# Autodesk Inventor assembly: 5
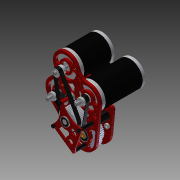
[picture p0: Inventor's stored thumbnail of the model, 180x180]
Saved by Autodesk Inventor 2013 (Build 170138000, 138)
## iProperties
Created: 2013-07-09
Part Number: 5
Document SubType Name: Assembly
Designer: mvarma
Author: mvarma
## Documents named in this file (40)
- C:\Users\mvarma\Desktop\GRT 2013-2014 Gearbox\Mark 5\Mark 5 Rendering Copy.iam
- C:\Users\mvarma\Desktop\GRT 2013-2014 Gearbox\Mark 5\Plates\Mounting Plate\Mounting Plate.ipt
- C:\Users\mvarma\Desktop\GRT 2013-2014 Gearbox\Mark 5\Plates\Cim Plate\Cim Plate.ipt
- C:\Users\mvarma\Desktop\GRT 2013-2014 Gearbox\Mark 5\Plates\Main Connecting Standoff Thick.ipt
- C:\Users\mvarma\Desktop\GRT 2013-2014 Gearbox\Mark 5\Plates\Main Connecting Standoff Thin.ipt
- C:\Users\mvarma\Desktop\GRT 2013-2014 Gearbox\Mark 5\Bearings\FR8-2RS.ipt
- C:\Users\mvarma\Desktop\GRT 2013-2014 Gearbox\Mark 5\Bearings\FR6-2RS.ipt
- C:\Users\mvarma\Desktop\GRT 2013-2014 Gearbox\Mark 5\Shafts\Cluster Shaft\15T 20DP - .375 Hex Bore.ipt
- C:\Users\mvarma\Desktop\GRT 2013-2014 Gearbox\Mark 5\Shafts\Cluster Shaft\28T 20DP - .375 Hex Bore.ipt
- C:\Users\mvarma\Desktop\GRT 2013-2014 Gearbox\Mark 5\Shafts\Cluster Shaft\Cluster Shaft Spacer.ipt
- C:\Users\mvarma\Desktop\GRT 2013-2014 Gearbox\Mark 5\Shafts\Cluster Shaft\Cluster Shaft.ipt
- C:\Users\mvarma\Desktop\GRT 2013-2014 Gearbox\Mark 5\Shafts\Cluster Shaft\48T 3mm GT2 - .375 Hex Broach - Hubless.ipt
- C:\Users\mvarma\Desktop\GRT 2013-2014 Gearbox\Mark 5\Shafts\Cluster Shaft\Flexible Shaft Coupler 6208K411.ipt
- C:\Users\mvarma\Desktop\GRT 2013-2014 Gearbox\Mark 5\Encoder\Encoder Mount.ipt
- C:\Users\mvarma\Desktop\GRT 2013-2014 Gearbox\Mark 5\Encoder\S4-120-250-N-S-B.ipt
- C:\Users\mvarma\Desktop\GRT 2013-2014 Gearbox\Mark 5\Shafts\Output Shaft\Output Shaft Hex Sleave.ipt
- C:\Users\mvarma\Desktop\GRT 2013-2014 Gearbox\Mark 5\Shafts\Output Shaft\Output Shaft Insert.ipt
- C:\Users\mvarma\Desktop\GRT 2013-2014 Gearbox\Mark 5\Shafts\Output Shaft\Output Shaft.ipt
- C:\Users\mvarma\Desktop\GRT 2013-2014 Gearbox\Mark 5\Shafts\Output Shaft\35T 20DP - .188 Ball Shifting Bore.ipt
- C:\Users\mvarma\Desktop\GRT 2013-2014 Gearbox\Mark 5\Shafts\Output Shaft\48T 20DP - .188 Ball Shifting Bore.ipt
- C:\Users\mvarma\Desktop\GRT 2013-2014 Gearbox\Mark 5\Bearings\Thrust Bearing Washer - .6250 Bore.ipt
- C:\Users\mvarma\Desktop\GRT 2013-2014 Gearbox\Mark 5\Bearings\R10-Open.ipt
- C:\Users\mvarma\Desktop\GRT 2013-2014 Gearbox\Mark 5\Shafts\Output Shaft\Shim 10 thou .500 Bore.ipt
- C:\Users\mvarma\Desktop\GRT 2013-2014 Gearbox\Mark 5\Shafts\Output Shaft\Shim 10 thou .625 Bore.ipt
- C:\Users\mvarma\Desktop\GRT 2013-2014 Gearbox\Mark 5\Plates\Mounting Plate\10-32 Clinch Style Pem Nut .091 Minimum Panel Thickness.ipt
- C:\Users\mvarma\Desktop\GRT 2013-2014 Gearbox\Mark 5\Plates\Mounting Plate\.25-20 Clinch Style Pem Nut .125 Minimum Panel Thickness.ipt
- C:\Users\mvarma\Desktop\GRT 2013-2014 Gearbox\Mark 5\Motors\CIM Can.ipt
- C:\Users\mvarma\Desktop\GRT 2013-2014 Gearbox\Mark 5\Motors\Rotor.ipt
- C:\Users\mvarma\Desktop\GRT 2013-2014 Gearbox\Mark 5\Motors\Mini CIM Can.ipt
- C:\Users\mvarma\Desktop\GRT 2013-2014 Gearbox\Mark 5\Pulleys\16T 3mm GT2 - 8mm Key Broach.ipt
- C:\Users\mvarma\Desktop\GRT 2013-2014 Gearbox\Mark 5\Belts\267 mm Belt.ipt
- C:\Users\mvarma\Desktop\GRT 2013-2014 Gearbox\Mark 5\Belts\285 mm Belt.ipt
- C:\Users\mvarma\Desktop\GRT 2013-2014 Gearbox\Mark 5\Plates\Tensioning Shaft.ipt
- C:\Users\mvarma\Desktop\GRT 2013-2014 Gearbox\Mark 5\Plates\Belt Shaft Spacer 2.ipt
- C:\Users\mvarma\Desktop\GRT 2013-2014 Gearbox\Mark 5\Bearings\R4-2RS.ipt
- C:\Users\mvarma\Desktop\GRT 2013-2014 Gearbox\Mark 5\Shafts\Cluster Shaft\Shim 10 thou .375 Bore.ipt
- C:\Users\mvarma\Desktop\GRT 2013-2014 Gearbox\Mark 5\Plates\Pnuematic Plate.ipt
- C:\Users\mvarma\Desktop\GRT 2013-2014 Gearbox\Mark 5\Plates\Supporting Plate Standoff Long.ipt
- C:\Users\mvarma\Desktop\GRT 2013-2014 Gearbox\Mark 5\Plates\Supporting Plate Standoff Short.ipt
- C:\Users\mvarma\Desktop\GRT 2013-2014 Gearbox\Mark 5\Bolts\Socket Head Cap Screw 10-32 Thread 3.000 Length.ipt
## Components (57 placed, 39 different names)
1. Mounting Plate:1 — Mate:1, Mate:2, Mate:3, Mate:5, Mate:11, Mate:13, Mate:15, Mate:16, Mate:17, Mate:18, Mate:52, Mate:53, Mate:54, Mate:76, Mate:77, Mate:78, Mate:79, Mate:80, Mate:81, Mate:82, Mate:83, Mate:101, Mate:102
2. Cim Plate:1 — Mate:7, Mate:8, Mate:9, Mate:12, Mate:14, Mate:19, Mate:86, Mate:87, Mate:88, Mate:89, Mate:90, Mate:91, Mate:96, Mate:97, Mate:98, Mate:115, Mate:116, Mate:124, Mate:125, Mate:126, Mate:130, Mate:131, Mate:132, Mate:133, Mate:134, Mate:135
3. Main Connecting Standoff Thick:1 — Mate:5, Mate:8, Mate:18
4. Main Connecting Standoff Thick:2 — Mate:3, Mate:7, Mate:17, Mate:19
5. Main Connecting Standoff Thin:1 — Mate:1, Mate:2, Mate:9
6. FR8-2RS:1 — Mate:12, Mate:14, Mate:55, Mate:75
7. FR8-2RS:2 — Mate:11, Mate:13
8. FR6-2RS:1 — Mate:15, Mate:16, Mate:33
9. 15T 20DP - .375 Hex Bore:1 — Mate:34, Mate:36, Mate:45, Mate:144
10. 28T 20DP - .375 Hex Bore:1 — Mate:34, Mate:37, Mate:38, Mate:45
11. Cluster Shaft Spacer:1 — Mate:30, Mate:31, Mate:33, Mate:38
12. Cluster Shaft:1 — Mate:30, Mate:31, Mate:36, Mate:37, Mate:39, Mate:40, Mate:41, Mate:42, Mate:44, Mate:48, Mate:49, Mate:121, Mate:123
13. 48T 3mm GT2 - .375 Hex Broach - Hubless:1 — Mate:39, Mate:41, Mate:43, Mate:44, Mate:104, Mate:106
14. 48T 3mm GT2 - .375 Hex Broach - Hubless:2 — Mate:40, Mate:42, Mate:43, Mate:108, Mate:122
15. Flexible Shaft Coupler 6208K411:1 — Mate:48, Mate:49
16. Encoder Mount:1 — Mate:50, Mate:51, Mate:52, Mate:53, Mate:54
17. S4-120-250-N-S-B:1 — Mate:50, Mate:51
18. Output Shaft Hex Sleave:1 — Mate:58, Mate:59, Flush:1
19. Output Shaft Insert:1 — Mate:56, Mate:57
20. Output Shaft:1 — Mate:55, Mate:56, Mate:57, Mate:58, Mate:59, Flush:1, Mate:61, Mate:66, Mate:67, Mate:70, Flush:2, Mate:72, Mate:73, Mate:75
21. 35T 20DP - .188 Ball Shifting Bore:1 — Mate:60, Mate:61, Mate:64, Mate:65, Mate:68
22. 48T 20DP - .188 Ball Shifting Bore:1 — Mate:60, Mate:62, Mate:63, Mate:69
23. Thrust Bearing Washer - .6250 Bore:1 — Mate:67, Mate:69, Mate:71
24. Thrust Bearing Washer - .6250 Bore:2 — Mate:66, Mate:68, Mate:74
25. R10-Open:1 — Mate:62, Mate:63, Mate:74
26. R10-Open:2 — Mate:64, Mate:65
27. Shim 10 thou .500 Bore:1 — Mate:72, Mate:73
28. Shim 10 thou .625 Bore:1 — Mate:70, Mate:71, Flush:2
29. 10-32 Clinch Style Pem Nut .091 Minimum Panel Thickness:1 — Mate:77, Mate:80
30. 10-32 Clinch Style Pem Nut .091 Minimum Panel Thickness:2 — Mate:78, Mate:81
31. 10-32 Clinch Style Pem Nut .091 Minimum Panel Thickness:3 — Mate:76, Mate:79
32. .25-20 Clinch Style Pem Nut .125 Minimum Panel Thickness:1 — Mate:82, Mate:101
33. .25-20 Clinch Style Pem Nut .125 Minimum Panel Thickness:2 — Mate:83, Mate:102
34. CIM Can:1 — Mate:88, Mate:89, Mate:90, Mate:94, Mate:95
35. CIM Can:2 — Mate:86, Mate:87, Mate:91, Mate:92, Mate:93
36. Rotor:1 — Mate:94, Mate:95, Mate:105, Mate:109
37. Rotor:2 — Mate:92, Mate:93, Mate:103
38. Rotor:3 — Mate:99, Mate:100, Mate:107, Mate:112
39. Mini CIM Can:1 — Mate:96, Mate:97, Mate:98, Mate:99, Mate:100
40. 16T 3mm GT2 - 8mm Key Broach:1 — Mate:105, Mate:106, Flush:3
41. 16T 3mm GT2 - 8mm Key Broach:2 — Mate:107, Mate:108, Mate:113
42. 16T 3mm GT2 - 8mm Key Broach:3 — Mate:103, Mate:104
43. 267 mm Belt:1 — Mate:109, Flush:3, Mate:143
44. 285 mm Belt:1 — Mate:112, Mate:113, Mate:142
45. Tensioning Shaft:1 — Mate:114, Flush:4, Mate:115, Mate:116, Mate:119, Mate:120
46. Belt Shaft Spacer 2:1 — Mate:114, Flush:4
47. R4-2RS:1 — Mate:117, Mate:118, Mate:119
48. R4-2RS:2 — Mate:117, Mate:118, Mate:120
49. Shim 10 thou .375 Bore:1 — Mate:121, Mate:122, Mate:129
50. Pnuematic Plate:1 — Mate:123, Mate:124, Mate:125, Mate:126, Mate:127, Mate:128, Mate:136, Mate:137, Mate:138, Mate:139, Mate:140, Mate:141, Mate:142, Mate:143, Mate:144
51. FR6-2RS:2 — Mate:127, Mate:128, Mate:129
52. Supporting Plate Standoff Long:1 — Mate:131, Mate:132
53. Supporting Plate Standoff Long:2 — Mate:130, Mate:133
54. Supporting Plate Standoff Short:1 — Mate:134, Mate:135
55. Socket Head Cap Screw 10-32 Thread 3.000 Length:1 — Mate:138, Mate:141
56. Socket Head Cap Screw 10-32 Thread 3.000 Length:2 — Mate:137, Mate:140
57. Socket Head Cap Screw 10-32 Thread 3.000 Length:3 — Mate:136, Mate:139
## Relationships (127: Mate 123, Flush 4)
- Mate:1: Mounting Plate:1 ↔ Main Connecting Standoff Thin:1
- Mate:2: Mounting Plate:1 ↔ Main Connecting Standoff Thin:1
- Mate:3: Mounting Plate:1 ↔ Main Connecting Standoff Thick:2
- Mate:5: Mounting Plate:1 ↔ Main Connecting Standoff Thick:1
- Mate:7: Cim Plate:1 ↔ Main Connecting Standoff Thick:2
- Mate:8: Cim Plate:1 ↔ Main Connecting Standoff Thick:1
- Mate:9: Cim Plate:1 ↔ Main Connecting Standoff Thin:1
- Mate:11: Mounting Plate:1 ↔ FR8-2RS:2
- Mate:12: Cim Plate:1 ↔ FR8-2RS:1
- Mate:13: Mounting Plate:1 ↔ FR8-2RS:2
- Mate:14: Cim Plate:1 ↔ FR8-2RS:1
- Mate:15: Mounting Plate:1 ↔ FR6-2RS:1
- Mate:16: Mounting Plate:1 ↔ FR6-2RS:1
- Mate:17: Mounting Plate:1 ↔ Main Connecting Standoff Thick:2
- Mate:18: Mounting Plate:1 ↔ Main Connecting Standoff Thick:1
- Mate:19: Cim Plate:1 ↔ Main Connecting Standoff Thick:2
- Mate:30: Cluster Shaft Spacer:1 ↔ Cluster Shaft:1
- Mate:31: Cluster Shaft Spacer:1 ↔ Cluster Shaft:1
- Mate:33: FR6-2RS:1 ↔ Cluster Shaft Spacer:1
- Mate:34: 15T 20DP - .375 Hex Bore:1 ↔ 28T 20DP - .375 Hex Bore:1
- Mate:36: 15T 20DP - .375 Hex Bore:1 ↔ Cluster Shaft:1
- Mate:37: 28T 20DP - .375 Hex Bore:1 ↔ Cluster Shaft:1
- Mate:38: 28T 20DP - .375 Hex Bore:1 ↔ Cluster Shaft Spacer:1
- Mate:39: Cluster Shaft:1 ↔ 48T 3mm GT2 - .375 Hex Broach - Hubless:1
- Mate:40: Cluster Shaft:1 ↔ 48T 3mm GT2 - .375 Hex Broach - Hubless:2
- Mate:41: Cluster Shaft:1 ↔ 48T 3mm GT2 - .375 Hex Broach - Hubless:1
- Mate:42: Cluster Shaft:1 ↔ 48T 3mm GT2 - .375 Hex Broach - Hubless:2
- Mate:43: 48T 3mm GT2 - .375 Hex Broach - Hubless:1 ↔ 48T 3mm GT2 - .375 Hex Broach - Hubless:2
- Mate:44: Cluster Shaft:1 ↔ 48T 3mm GT2 - .375 Hex Broach - Hubless:1
- Mate:45: 15T 20DP - .375 Hex Bore:1 ↔ 28T 20DP - .375 Hex Bore:1
- Mate:48: Cluster Shaft:1 ↔ Flexible Shaft Coupler 6208K411:1
- Mate:49: Cluster Shaft:1 ↔ Flexible Shaft Coupler 6208K411:1
- Mate:50: Encoder Mount:1 ↔ S4-120-250-N-S-B:1
- Mate:51: Encoder Mount:1 ↔ S4-120-250-N-S-B:1
- Mate:52: Mounting Plate:1 ↔ Encoder Mount:1
- Mate:53: Mounting Plate:1 ↔ Encoder Mount:1
- Mate:54: Mounting Plate:1 ↔ Encoder Mount:1
- Mate:55: FR8-2RS:1 ↔ Output Shaft:1
- Mate:56: Output Shaft Insert:1 ↔ Output Shaft:1
- Mate:57: Output Shaft Insert:1 ↔ Output Shaft:1
- Mate:58: Output Shaft Hex Sleave:1 ↔ Output Shaft:1
- Mate:59: Output Shaft Hex Sleave:1 ↔ Output Shaft:1
- Flush:1: Output Shaft Hex Sleave:1 ↔ Output Shaft:1
- Mate:60: 35T 20DP - .188 Ball Shifting Bore:1 ↔ 48T 20DP - .188 Ball Shifting Bore:1
- Mate:61: Output Shaft:1 ↔ 35T 20DP - .188 Ball Shifting Bore:1
- Mate:62: 48T 20DP - .188 Ball Shifting Bore:1 ↔ R10-Open:1
- Mate:63: 48T 20DP - .188 Ball Shifting Bore:1 ↔ R10-Open:1
- Mate:64: 35T 20DP - .188 Ball Shifting Bore:1 ↔ R10-Open:2
- Mate:65: 35T 20DP - .188 Ball Shifting Bore:1 ↔ R10-Open:2
- Mate:66: Output Shaft:1 ↔ Thrust Bearing Washer - .6250 Bore:2
- Mate:67: Output Shaft:1 ↔ Thrust Bearing Washer - .6250 Bore:1
- Mate:68: 35T 20DP - .188 Ball Shifting Bore:1 ↔ Thrust Bearing Washer - .6250 Bore:2
- Mate:69: 48T 20DP - .188 Ball Shifting Bore:1 ↔ Thrust Bearing Washer - .6250 Bore:1
- Mate:70: Output Shaft:1 ↔ Shim 10 thou .625 Bore:1
- Mate:71: Thrust Bearing Washer - .6250 Bore:1 ↔ Shim 10 thou .625 Bore:1
- Flush:2: Output Shaft:1 ↔ Shim 10 thou .625 Bore:1
- Mate:72: Output Shaft:1 ↔ Shim 10 thou .500 Bore:1
- Mate:73: Output Shaft:1 ↔ Shim 10 thou .500 Bore:1
- Mate:74: Thrust Bearing Washer - .6250 Bore:2 ↔ R10-Open:1
- Mate:75: FR8-2RS:1 ↔ Output Shaft:1
- Mate:76: Mounting Plate:1 ↔ 10-32 Clinch Style Pem Nut .091 Minimum Panel Thickness:3
- Mate:77: Mounting Plate:1 ↔ 10-32 Clinch Style Pem Nut .091 Minimum Panel Thickness:1
- Mate:78: Mounting Plate:1 ↔ 10-32 Clinch Style Pem Nut .091 Minimum Panel Thickness:2
- Mate:79: Mounting Plate:1 ↔ 10-32 Clinch Style Pem Nut .091 Minimum Panel Thickness:3
- Mate:80: Mounting Plate:1 ↔ 10-32 Clinch Style Pem Nut .091 Minimum Panel Thickness:1
- Mate:81: Mounting Plate:1 ↔ 10-32 Clinch Style Pem Nut .091 Minimum Panel Thickness:2
- Mate:82: Mounting Plate:1 ↔ .25-20 Clinch Style Pem Nut .125 Minimum Panel Thickness:1
- Mate:83: Mounting Plate:1 ↔ .25-20 Clinch Style Pem Nut .125 Minimum Panel Thickness:2
- Mate:86: Cim Plate:1 ↔ CIM Can:2
- Mate:87: Cim Plate:1 ↔ CIM Can:2
- Mate:88: Cim Plate:1 ↔ CIM Can:1
- Mate:89: Cim Plate:1 ↔ CIM Can:1
- Mate:90: Cim Plate:1 ↔ CIM Can:1
- Mate:91: Cim Plate:1 ↔ CIM Can:2
- Mate:92: CIM Can:2 ↔ Rotor:2
- Mate:93: CIM Can:2 ↔ Rotor:2
- Mate:94: CIM Can:1 ↔ Rotor:1
- Mate:95: CIM Can:1 ↔ Rotor:1
- Mate:96: Cim Plate:1 ↔ Mini CIM Can:1
- Mate:97: Cim Plate:1 ↔ Mini CIM Can:1
- Mate:98: Cim Plate:1 ↔ Mini CIM Can:1
- Mate:99: Rotor:3 ↔ Mini CIM Can:1
- Mate:100: Rotor:3 ↔ Mini CIM Can:1
- Mate:101: Mounting Plate:1 ↔ .25-20 Clinch Style Pem Nut .125 Minimum Panel Thickness:1
- Mate:102: Mounting Plate:1 ↔ .25-20 Clinch Style Pem Nut .125 Minimum Panel Thickness:2
- Mate:103: Rotor:2 ↔ 16T 3mm GT2 - 8mm Key Broach:3
- Mate:104: 48T 3mm GT2 - .375 Hex Broach - Hubless:1 ↔ 16T 3mm GT2 - 8mm Key Broach:3
- Mate:105: Rotor:1 ↔ 16T 3mm GT2 - 8mm Key Broach:1
- Mate:106: 48T 3mm GT2 - .375 Hex Broach - Hubless:1 ↔ 16T 3mm GT2 - 8mm Key Broach:1
- Mate:107: Rotor:3 ↔ 16T 3mm GT2 - 8mm Key Broach:2
- Mate:108: 48T 3mm GT2 - .375 Hex Broach - Hubless:2 ↔ 16T 3mm GT2 - 8mm Key Broach:2
- Mate:109: Rotor:1 ↔ 267 mm Belt:1
- Flush:3: 16T 3mm GT2 - 8mm Key Broach:1 ↔ 267 mm Belt:1
- Mate:112: Rotor:3 ↔ 285 mm Belt:1
- Mate:113: 16T 3mm GT2 - 8mm Key Broach:2 ↔ 285 mm Belt:1
- Mate:114: Tensioning Shaft:1 ↔ Belt Shaft Spacer 2:1
- Flush:4: Tensioning Shaft:1 ↔ Belt Shaft Spacer 2:1
- Mate:115: Cim Plate:1 ↔ Tensioning Shaft:1
- Mate:116: Cim Plate:1 ↔ Tensioning Shaft:1
- Mate:117: R4-2RS:1 ↔ R4-2RS:2
- Mate:118: R4-2RS:1 ↔ R4-2RS:2
- Mate:119: Tensioning Shaft:1 ↔ R4-2RS:1
- Mate:120: Tensioning Shaft:1 ↔ R4-2RS:2
- Mate:121: Cluster Shaft:1 ↔ Shim 10 thou .375 Bore:1
- Mate:122: 48T 3mm GT2 - .375 Hex Broach - Hubless:2 ↔ Shim 10 thou .375 Bore:1
- Mate:123: Cluster Shaft:1 ↔ Pnuematic Plate:1
- Mate:124: Cim Plate:1 ↔ Pnuematic Plate:1
- Mate:125: Cim Plate:1 ↔ Pnuematic Plate:1
- Mate:126: Cim Plate:1 ↔ Pnuematic Plate:1
- Mate:127: Pnuematic Plate:1 ↔ FR6-2RS:2
- Mate:128: Pnuematic Plate:1 ↔ FR6-2RS:2
- Mate:129: Shim 10 thou .375 Bore:1 ↔ FR6-2RS:2
- Mate:130: Cim Plate:1 ↔ Supporting Plate Standoff Long:2
- Mate:131: Cim Plate:1 ↔ Supporting Plate Standoff Long:1
- Mate:132: Cim Plate:1 ↔ Supporting Plate Standoff Long:1
- Mate:133: Cim Plate:1 ↔ Supporting Plate Standoff Long:2
- Mate:134: Cim Plate:1 ↔ Supporting Plate Standoff Short:1
- Mate:135: Cim Plate:1 ↔ Supporting Plate Standoff Short:1
- Mate:136: Pnuematic Plate:1 ↔ Socket Head Cap Screw 10-32 Thread 3.000 Length:3
- Mate:137: Pnuematic Plate:1 ↔ Socket Head Cap Screw 10-32 Thread 3.000 Length:2
- Mate:138: Pnuematic Plate:1 ↔ Socket Head Cap Screw 10-32 Thread 3.000 Length:1
- Mate:139: Pnuematic Plate:1 ↔ Socket Head Cap Screw 10-32 Thread 3.000 Length:3
- Mate:140: Pnuematic Plate:1 ↔ Socket Head Cap Screw 10-32 Thread 3.000 Length:2
- Mate:141: Pnuematic Plate:1 ↔ Socket Head Cap Screw 10-32 Thread 3.000 Length:1
- Mate:142: 285 mm Belt:1 ↔ Pnuematic Plate:1
- Mate:143: 267 mm Belt:1 ↔ Pnuematic Plate:1
- Mate:144: 15T 20DP - .375 Hex Bore:1 ↔ Pnuematic Plate:1
